# Autodesk Inventor assembly: 機体
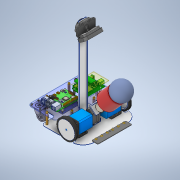
[picture p0: Inventor's stored thumbnail of the model, 180x180]
Saved by Autodesk Inventor 2020 (Build 240168000, 168)
## iProperties
Created: 2020-06-21
Part Number: 機体
Document SubType Name: Assembly
Designer: bsat3
Author: bsat3
## Documents named in this file (28)
- C:\Users\haya\Documents\Lecture\ロボット設計製作論４\2020\monotaro\IRC\機体.iam
- C:\Users\haya\Documents\Lecture\ロボット設計製作論４\2020\monotaro\IRC\知能ロボット\台車土台.ipt
- C:\Users\haya\Documents\Lecture\ロボット設計製作論４\2020\monotaro\IRC\モータ部分.iam
- C:\Users\haya\Documents\Lecture\ロボット設計製作論４\2020\monotaro\IRC\知能ロボット\知能ロボット吸引機構.iam
- C:\Users\haya\Documents\Lecture\ロボット設計製作論４\2020\monotaro\IRC\line_sensor.ipt
- C:\Users\haya\Documents\Lecture\ロボット設計製作論４\2020\monotaro\IRC\キャスタ.ipt
- C:\Users\haya\Documents\Lecture\ロボット設計製作論４\2020\monotaro\IRC\SBD-O3-25.ipt
- C:\Users\haya\Documents\Lecture\ロボット設計製作論４\2020\monotaro\IRC\arduino\arduino uno.iam
- C:\Users\haya\Documents\Lecture\ロボット設計製作論４\2020\monotaro\IRC\upper_frame.ipt
- C:\Users\haya\Documents\Lecture\ロボット設計製作論４\2020\monotaro\IRC\servo_motor\KRS2500_scale.ipt
- C:\Users\haya\Documents\Lecture\ロボット設計製作論４\2020\monotaro\IRC\fan_motor\Assembly 1.iam
- C:\Users\haya\Documents\Lecture\ロボット設計製作論４\2020\monotaro\IRC\arm.ipt
- C:\Users\haya\Documents\Lecture\ロボット設計製作論４\2020\monotaro\IRC\camera\CAMERA ASSEMBLY.iam
- C:\Users\haya\Documents\Lecture\ロボット設計製作論４\2020\monotaro\IRC\camera_stand.ipt
- C:\Users\haya\Documents\Lecture\ロボット設計製作論４\2020\monotaro\IRC\raspberrypi\Raspberry Pi 4 Model B.iam
- C:\Users\haya\Documents\Lecture\ロボット設計製作論４\2020\monotaro\IRC\battery_holder\1_5V_holder4AA.ipt
- C:\Users\haya\Documents\Lecture\ロボット設計製作論４\2020\monotaro\IRC\servo_arm.ipt
- C:\Users\haya\Documents\Lecture\ロボット設計製作論４\2020\monotaro\IRC\ball.ipt
- C:\Users\haya\Documents\Lecture\ロボット設計製作論４\2020\monotaro\IRC\servo_bracket.ipt
- C:\Users\haya\Documents\Lecture\ロボット設計製作論４\2020\monotaro\IRC\BOB-M3-2-3W.ipt
- C:\Users\haya\Documents\Lecture\ロボット設計製作論４\2020\monotaro\IRC\motor driver.ipt
- C:\Users\haya\Documents\Lecture\ロボット設計製作論４\2020\monotaro\IRC\shield.ipt
- C:\Users\haya\Documents\Lecture\ロボット設計製作論４\2020\monotaro\IRC\CSPELH-SUS-M3-5.ipt
- C:\Users\haya\Documents\Lecture\ロボット設計製作論４\2020\monotaro\IRC\CSPELH-SUS-M3-7.ipt
- C:\Users\haya\Documents\Lecture\ロボット設計製作論４\2020\monotaro\IRC\spacer_10mm.ipt
- C:\Users\haya\Documents\Lecture\ロボット設計製作論４\2020\monotaro\IRC\HNT1-ST-M3.ipt
- C:\Users\haya\Documents\Lecture\ロボット設計製作論４\2020\monotaro\IRC\CSPPN-ST-M3-6_203.ipt
- C:\Users\haya\Documents\Lecture\ロボット設計製作論４\2020\monotaro\IRC\E-6598.ipt
## Components (109 placed, 27 different names)
1. 台車土台:1 — メイト:3, フラッシュ:4, フラッシュ:5, メイト:5, メイト:6, メイト:7, メイト:8, 挿入:9, 挿入:10, 挿入:11, 挿入:12, 挿入:13, 挿入:14, フラッシュ:7, フラッシュ:8, メイト:13, メイト:18, フラッシュ:9, 挿入:32, 挿入:33, 挿入:42, 挿入:43, 挿入:48, 挿入:49, 挿入:50, 挿入:51, 挿入:52, 挿入:53, 挿入:54, 挿入:55, 挿入:56, 挿入:57, 挿入:58, 挿入:59, 挿入:60, 挿入:61, 挿入:62, 挿入:63, 挿入:64, 挿入:65, 挿入:66, 挿入:67, 挿入:68, 挿入:69, 挿入:70, 挿入:71, 挿入:72, 挿入:73, 挿入:74, 挿入:75
2. モータ部分:1 [sub-assembly] — フラッシュ:4, メイト:5, メイト:6
3. モータ部分:2 [sub-assembly] — フラッシュ:5, メイト:7, メイト:8
4. 知能ロボット吸引機構:1 [sub-assembly] — 挿入:24, 挿入:25, メイト:19, メイト:20
5. line_sensor:1 — 挿入:42, 挿入:43, 挿入:85, 挿入:86, 挿入:87, 挿入:88, 挿入:89, 挿入:90
6. キャスタ:1 — 挿入:15, 挿入:16, 挿入:34, 挿入:35, 挿入:36, 挿入:37
7. SBD-O3-25:1 — メイト:3, 挿入:9
8. arduino uno:1 [sub-assembly] — メイト:11, メイト:21, フラッシュ:10, フラッシュ:11, フラッシュ:16, フラッシュ:17, 挿入:81, 挿入:82, 挿入:83, 挿入:84
9. SBD-O3-25:2 — 挿入:10
10. SBD-O3-25:3 — 挿入:11
11. SBD-O3-25:4 — 挿入:12, メイト:10
12. SBD-O3-25:5 — 挿入:13
13. SBD-O3-25:6 — 挿入:14
14. upper_frame:1 — メイト:10, フラッシュ:7, 挿入:15, 挿入:16, 挿入:17, 挿入:18, フラッシュ:8, メイト:11, メイト:14, メイト:15, メイト:17, フラッシュ:16, フラッシュ:17, フラッシュ:18, フラッシュ:19, 挿入:91, 挿入:92, 挿入:93, 挿入:94, 挿入:95, 挿入:96, 挿入:97, 挿入:98, 挿入:99, 挿入:100, 挿入:101, 挿入:102, 挿入:103, 挿入:104, 挿入:105, 挿入:106, 挿入:107, 挿入:108, 挿入:109, 挿入:110, 挿入:111, 挿入:112
15. キャスタ:2 — 挿入:17, 挿入:18, 挿入:38, 挿入:39, 挿入:40, 挿入:41
16. KRS2500_scale:1 — 挿入:21, 挿入:26, 挿入:27
17. Assembly 1:1 [sub-assembly] — 挿入:19
18. arm:1 — 挿入:19, 挿入:22, 挿入:23, 挿入:24, 挿入:25
19. CAMERA ASSEMBLY:1 [sub-assembly] — メイト:16, メイト:24, 角度:1
20. camera_stand:1 — メイト:13, メイト:14, メイト:15, メイト:16, 挿入:44, 挿入:45, 挿入:46, 挿入:47, 挿入:113, 角度:1
21. Raspberry Pi 4 Model B:1 [sub-assembly] — メイト:17, フラッシュ:18, フラッシュ:19, 挿入:76, 挿入:77, 挿入:78, 挿入:79
22. 1_5V_holder4AA:1 — メイト:18, フラッシュ:9
23. servo_arm:1 — 挿入:21, 挿入:22, 挿入:23
24. ball:1 — メイト:19, メイト:20
25. servo_bracket:1 — 挿入:26, 挿入:27, 挿入:28, 挿入:29, 挿入:30, 挿入:31, 挿入:32, 挿入:33
26. BOB-M3-2-3W:1 — 挿入:28
27. BOB-M3-2-3W:2 — 挿入:29
28. BOB-M3-2-3W:3 — 挿入:30
29. BOB-M3-2-3W:4 — 挿入:31
30. BOB-M3-2-3W:5 — 挿入:34
31. BOB-M3-2-3W:6 — 挿入:35
32. BOB-M3-2-3W:7 — 挿入:36
33. BOB-M3-2-3W:8 — 挿入:37
34. BOB-M3-2-3W:9 — 挿入:38
35. BOB-M3-2-3W:10 — 挿入:39
36. BOB-M3-2-3W:11 — 挿入:41
37. BOB-M3-2-3W:12 — 挿入:40
38. motor driver:1 — メイト:23, フラッシュ:13, フラッシュ:15
39. motor driver:2 — メイト:22, フラッシュ:12, フラッシュ:14
40. shield:1 — メイト:21, フラッシュ:10, フラッシュ:11, メイト:22, フラッシュ:12, メイト:23, フラッシュ:13, フラッシュ:14, フラッシュ:15
41. BOB-M3-2-3W:13 — 挿入:44
42. BOB-M3-2-3W:14 — 挿入:45
43. BOB-M3-2-3W:15 — 挿入:46
44. BOB-M3-2-3W:16 — 挿入:47
45. CSPELH-SUS-M3-5:1 — 挿入:48
46. CSPELH-SUS-M3-5:2 — 挿入:49
47. CSPELH-SUS-M3-5:3 — 挿入:50
48. CSPELH-SUS-M3-5:4 — 挿入:51
49. CSPELH-SUS-M3-7:1 — 挿入:52
50. CSPELH-SUS-M3-7:2 — 挿入:53
51. CSPELH-SUS-M3-7:3 — 挿入:54
52. CSPELH-SUS-M3-7:4 — 挿入:55
53. CSPELH-SUS-M3-7:5 — 挿入:56
54. CSPELH-SUS-M3-7:6 — 挿入:58
55. CSPELH-SUS-M3-7:7 — 挿入:59
56. CSPELH-SUS-M3-7:8 — 挿入:57
57. CSPELH-SUS-M3-7:10 — 挿入:62
58. CSPELH-SUS-M3-7:11 — 挿入:61
59. CSPELH-SUS-M3-7:12 — 挿入:60
60. CSPELH-SUS-M3-7:13 — 挿入:63
61. CSPELH-SUS-M3-7:14 — 挿入:64
62. CSPELH-SUS-M3-7:15 — 挿入:65
63. CSPELH-SUS-M3-7:16 — 挿入:67
64. CSPELH-SUS-M3-7:17 — 挿入:66
65. CSPELH-SUS-M3-7:18 — 挿入:68
66. CSPELH-SUS-M3-7:19 — 挿入:72
67. CSPELH-SUS-M3-7:20 — 挿入:70
68. CSPELH-SUS-M3-7:21 — 挿入:71
69. CSPELH-SUS-M3-7:22 — 挿入:69
70. CSPELH-SUS-M3-7:23 — 挿入:75
71. CSPELH-SUS-M3-7:24 — 挿入:74
72. CSPELH-SUS-M3-7:25 — 挿入:73
73. spacer_10mm:1 — 挿入:78
74. spacer_10mm:2 — 挿入:79
75. spacer_10mm:3 — 挿入:77
76. spacer_10mm:4 — 挿入:76
77. spacer_10mm:6 — 挿入:81
78. spacer_10mm:7 — 挿入:83
79. spacer_10mm:8 — 挿入:82
80. spacer_10mm:9 — 挿入:84
81. HNT1-ST-M3:1 — 挿入:85
82. HNT1-ST-M3:2 — 挿入:90
83. HNT1-ST-M3:3 — 挿入:89
84. HNT1-ST-M3:4 — 挿入:88
85. HNT1-ST-M3:5 — 挿入:87
86. HNT1-ST-M3:6 — 挿入:86
87. HNT1-ST-M3:7 — 挿入:96
88. HNT1-ST-M3:8 — 挿入:94
89. HNT1-ST-M3:9 — 挿入:93
90. HNT1-ST-M3:10 — 挿入:95
91. HNT1-ST-M3:11 — 挿入:92
92. HNT1-ST-M3:12 — 挿入:91
93. CSPPN-ST-M3-6_203:1 — 挿入:97
94. CSPPN-ST-M3-6_203:2 — 挿入:98
95. CSPPN-ST-M3-6_203:3 — 挿入:99
96. CSPPN-ST-M3-6_203:4 — 挿入:100
97. CSPPN-ST-M3-6_203:5 — 挿入:101
98. CSPPN-ST-M3-6_203:6 — 挿入:102
99. CSPPN-ST-M3-6_203:7 — 挿入:103
100. CSPPN-ST-M3-6_203:8 — 挿入:104
101. CSPPN-ST-M3-6_203:9 — 挿入:105
102. CSPPN-ST-M3-6_203:10 — 挿入:108
103. CSPPN-ST-M3-6_203:11 — 挿入:107
104. CSPPN-ST-M3-6_203:12 — 挿入:106
105. CSPPN-ST-M3-6_203:13 — 挿入:109
106. CSPPN-ST-M3-6_203:14 — 挿入:110
107. CSPPN-ST-M3-6_203:15 — 挿入:111
108. CSPPN-ST-M3-6_203:16 — 挿入:112
109. E-6598:1 — 挿入:113, メイト:24
## Relationships (138: Insert 103, Mate 19, Flush 15, Angle 1)
- メイト:3 [Mate]: 台車土台:1 ↔ SBD-O3-25:1
- フラッシュ:4 [Flush]: 台車土台:1 ↔ モータ部分:1
- フラッシュ:5 [Flush]: 台車土台:1 ↔ モータ部分:2
- メイト:5 [Mate]: 台車土台:1 ↔ モータ部分:1
- メイト:6 [Mate] (-60 mm): 台車土台:1 ↔ モータ部分:1
- メイト:7 [Mate]: 台車土台:1 ↔ モータ部分:2
- メイト:8 [Mate] (-60 mm): 台車土台:1 ↔ モータ部分:2
- 挿入:9 [Insert]: 台車土台:1 ↔ SBD-O3-25:1
- 挿入:10 [Insert]: 台車土台:1 ↔ SBD-O3-25:2
- 挿入:11 [Insert]: 台車土台:1 ↔ SBD-O3-25:3
- 挿入:12 [Insert]: 台車土台:1 ↔ SBD-O3-25:4
- 挿入:13 [Insert]: 台車土台:1 ↔ SBD-O3-25:5
- 挿入:14 [Insert]: 台車土台:1 ↔ SBD-O3-25:6
- メイト:10 [Mate]: SBD-O3-25:4 ↔ upper_frame:1
- フラッシュ:7 [Flush]: 台車土台:1 ↔ upper_frame:1
- 挿入:15 [Insert]: キャスタ:1 ↔ upper_frame:1
- 挿入:16 [Insert]: キャスタ:1 ↔ upper_frame:1
- 挿入:17 [Insert]: upper_frame:1 ↔ キャスタ:2
- 挿入:18 [Insert]: upper_frame:1 ↔ キャスタ:2
- フラッシュ:8 [Flush]: 台車土台:1 ↔ upper_frame:1
- メイト:11 [Mate] (10 mm): arduino uno:1 ↔ upper_frame:1
- 挿入:19 [Insert]: Assembly 1:1 ↔ arm:1
- メイト:13 [Mate]: 台車土台:1 ↔ camera_stand:1
- メイト:14 [Mate]: upper_frame:1 ↔ camera_stand:1
- メイト:15 [Mate]: upper_frame:1 ↔ camera_stand:1
- メイト:16 [Mate]: CAMERA ASSEMBLY:1 ↔ camera_stand:1
- メイト:17 [Mate] (10 mm): upper_frame:1 ↔ Raspberry Pi 4 Model B:1
- メイト:18 [Mate]: 台車土台:1 ↔ 1_5V_holder4AA:1
- フラッシュ:9 [Flush]: 台車土台:1 ↔ 1_5V_holder4AA:1
- 挿入:21 [Insert] (3 mm): KRS2500_scale:1 ↔ servo_arm:1
- 挿入:22 [Insert]: arm:1 ↔ servo_arm:1
- 挿入:23 [Insert]: arm:1 ↔ servo_arm:1
- 挿入:24 [Insert]: 知能ロボット吸引機構:1 ↔ arm:1
- 挿入:25 [Insert]: 知能ロボット吸引機構:1 ↔ arm:1
- メイト:19 [Mate]: 知能ロボット吸引機構:1 ↔ ball:1
- メイト:20 [Mate] (16 mm): 知能ロボット吸引機構:1 ↔ ball:1
- 挿入:26 [Insert]: KRS2500_scale:1 ↔ servo_bracket:1
- 挿入:27 [Insert]: KRS2500_scale:1 ↔ servo_bracket:1
- 挿入:28 [Insert]: servo_bracket:1 ↔ BOB-M3-2-3W:1
- 挿入:29 [Insert]: servo_bracket:1 ↔ BOB-M3-2-3W:2
- 挿入:30 [Insert]: servo_bracket:1 ↔ BOB-M3-2-3W:3
- 挿入:31 [Insert]: servo_bracket:1 ↔ BOB-M3-2-3W:4
- 挿入:32 [Insert]: 台車土台:1 ↔ servo_bracket:1
- 挿入:33 [Insert]: 台車土台:1 ↔ servo_bracket:1
- 挿入:34 [Insert]: キャスタ:1 ↔ BOB-M3-2-3W:5
- 挿入:35 [Insert]: キャスタ:1 ↔ BOB-M3-2-3W:6
- 挿入:36 [Insert]: キャスタ:1 ↔ BOB-M3-2-3W:7
- 挿入:37 [Insert]: キャスタ:1 ↔ BOB-M3-2-3W:8
- 挿入:38 [Insert]: キャスタ:2 ↔ BOB-M3-2-3W:9
- 挿入:39 [Insert]: キャスタ:2 ↔ BOB-M3-2-3W:10
- 挿入:40 [Insert]: キャスタ:2 ↔ BOB-M3-2-3W:12
- 挿入:41 [Insert]: キャスタ:2 ↔ BOB-M3-2-3W:11
- 挿入:42 [Insert]: 台車土台:1 ↔ line_sensor:1
- 挿入:43 [Insert]: 台車土台:1 ↔ line_sensor:1
- メイト:21 [Mate] (3 mm): arduino uno:1 ↔ shield:1
- フラッシュ:10 [Flush]: arduino uno:1 ↔ shield:1
- フラッシュ:11 [Flush]: arduino uno:1 ↔ shield:1
- メイト:22 [Mate] (10 mm): motor driver:2 ↔ shield:1
- フラッシュ:12 [Flush] (4 mm): motor driver:2 ↔ shield:1
- メイト:23 [Mate] (10 mm): motor driver:1 ↔ shield:1
- フラッシュ:13 [Flush] (26 mm): motor driver:1 ↔ shield:1
- フラッシュ:14 [Flush] (6 mm): motor driver:2 ↔ shield:1
- フラッシュ:15 [Flush] (6 mm): motor driver:1 ↔ shield:1
- フラッシュ:16 [Flush] (14 mm): arduino uno:1 ↔ upper_frame:1
- フラッシュ:17 [Flush] (22 mm): arduino uno:1 ↔ upper_frame:1
- フラッシュ:18 [Flush] (30 mm): upper_frame:1 ↔ Raspberry Pi 4 Model B:1
- フラッシュ:19 [Flush] (20 mm): upper_frame:1 ↔ Raspberry Pi 4 Model B:1
- 挿入:44 [Insert]: camera_stand:1 ↔ BOB-M3-2-3W:13
- 挿入:45 [Insert]: camera_stand:1 ↔ BOB-M3-2-3W:14
- 挿入:46 [Insert]: camera_stand:1 ↔ BOB-M3-2-3W:15
- 挿入:47 [Insert]: camera_stand:1 ↔ BOB-M3-2-3W:16
- 挿入:48 [Insert]: 台車土台:1 ↔ CSPELH-SUS-M3-5:1
- 挿入:49 [Insert]: 台車土台:1 ↔ CSPELH-SUS-M3-5:2
- 挿入:50 [Insert]: 台車土台:1 ↔ CSPELH-SUS-M3-5:3
- 挿入:51 [Insert]: 台車土台:1 ↔ CSPELH-SUS-M3-5:4
- 挿入:52 [Insert]: 台車土台:1 ↔ CSPELH-SUS-M3-7:1
- 挿入:53 [Insert]: 台車土台:1 ↔ CSPELH-SUS-M3-7:2
- 挿入:54 [Insert]: 台車土台:1 ↔ CSPELH-SUS-M3-7:3
- 挿入:55 [Insert]: 台車土台:1 ↔ CSPELH-SUS-M3-7:4
- 挿入:56 [Insert]: 台車土台:1 ↔ CSPELH-SUS-M3-7:5
- 挿入:57 [Insert]: 台車土台:1 ↔ CSPELH-SUS-M3-7:8
- 挿入:58 [Insert]: 台車土台:1 ↔ CSPELH-SUS-M3-7:6
- 挿入:59 [Insert]: 台車土台:1 ↔ CSPELH-SUS-M3-7:7
- 挿入:60 [Insert]: 台車土台:1 ↔ CSPELH-SUS-M3-7:12
- 挿入:61 [Insert]: 台車土台:1 ↔ CSPELH-SUS-M3-7:11
- 挿入:62 [Insert]: 台車土台:1 ↔ CSPELH-SUS-M3-7:10
- 挿入:63 [Insert]: 台車土台:1 ↔ CSPELH-SUS-M3-7:13
- 挿入:64 [Insert]: 台車土台:1 ↔ CSPELH-SUS-M3-7:14
- 挿入:65 [Insert]: 台車土台:1 ↔ CSPELH-SUS-M3-7:15
- 挿入:66 [Insert]: 台車土台:1 ↔ CSPELH-SUS-M3-7:17
- 挿入:67 [Insert]: 台車土台:1 ↔ CSPELH-SUS-M3-7:16
- 挿入:68 [Insert]: 台車土台:1 ↔ CSPELH-SUS-M3-7:18
- 挿入:69 [Insert]: 台車土台:1 ↔ CSPELH-SUS-M3-7:22
- 挿入:70 [Insert]: 台車土台:1 ↔ CSPELH-SUS-M3-7:20
- 挿入:71 [Insert]: 台車土台:1 ↔ CSPELH-SUS-M3-7:21
- 挿入:72 [Insert]: 台車土台:1 ↔ CSPELH-SUS-M3-7:19
- 挿入:73 [Insert]: 台車土台:1 ↔ CSPELH-SUS-M3-7:25
- 挿入:74 [Insert]: 台車土台:1 ↔ CSPELH-SUS-M3-7:24
- 挿入:75 [Insert]: 台車土台:1 ↔ CSPELH-SUS-M3-7:23
- 挿入:76 [Insert]: Raspberry Pi 4 Model B:1 ↔ spacer_10mm:4
- 挿入:77 [Insert]: Raspberry Pi 4 Model B:1 ↔ spacer_10mm:3
- 挿入:78 [Insert]: Raspberry Pi 4 Model B:1 ↔ spacer_10mm:1
- 挿入:79 [Insert]: Raspberry Pi 4 Model B:1 ↔ spacer_10mm:2
- 挿入:81 [Insert]: arduino uno:1 ↔ spacer_10mm:6
- 挿入:82 [Insert]: arduino uno:1 ↔ spacer_10mm:8
- 挿入:83 [Insert]: arduino uno:1 ↔ spacer_10mm:7
- 挿入:84 [Insert]: arduino uno:1 ↔ spacer_10mm:9
- 挿入:85 [Insert]: line_sensor:1 ↔ HNT1-ST-M3:1
- 挿入:86 [Insert]: line_sensor:1 ↔ HNT1-ST-M3:6
- 挿入:87 [Insert]: line_sensor:1 ↔ HNT1-ST-M3:5
- 挿入:88 [Insert]: line_sensor:1 ↔ HNT1-ST-M3:4
- 挿入:89 [Insert]: line_sensor:1 ↔ HNT1-ST-M3:3
- 挿入:90 [Insert]: line_sensor:1 ↔ HNT1-ST-M3:2
- 挿入:91 [Insert]: upper_frame:1 ↔ HNT1-ST-M3:12
- 挿入:92 [Insert]: upper_frame:1 ↔ HNT1-ST-M3:11
- 挿入:93 [Insert]: upper_frame:1 ↔ HNT1-ST-M3:9
- 挿入:94 [Insert]: upper_frame:1 ↔ HNT1-ST-M3:8
- 挿入:95 [Insert]: upper_frame:1 ↔ HNT1-ST-M3:10
- 挿入:96 [Insert]: upper_frame:1 ↔ HNT1-ST-M3:7
- 挿入:97 [Insert]: upper_frame:1 ↔ CSPPN-ST-M3-6_203:1
- 挿入:98 [Insert]: upper_frame:1 ↔ CSPPN-ST-M3-6_203:2
- 挿入:99 [Insert]: upper_frame:1 ↔ CSPPN-ST-M3-6_203:3
- 挿入:100 [Insert]: upper_frame:1 ↔ CSPPN-ST-M3-6_203:4
- 挿入:101 [Insert]: upper_frame:1 ↔ CSPPN-ST-M3-6_203:5
- 挿入:102 [Insert]: upper_frame:1 ↔ CSPPN-ST-M3-6_203:6
- 挿入:103 [Insert]: upper_frame:1 ↔ CSPPN-ST-M3-6_203:7
- 挿入:104 [Insert]: upper_frame:1 ↔ CSPPN-ST-M3-6_203:8
- 挿入:105 [Insert]: upper_frame:1 ↔ CSPPN-ST-M3-6_203:9
- 挿入:106 [Insert]: upper_frame:1 ↔ CSPPN-ST-M3-6_203:12
- 挿入:107 [Insert]: upper_frame:1 ↔ CSPPN-ST-M3-6_203:11
- 挿入:108 [Insert]: upper_frame:1 ↔ CSPPN-ST-M3-6_203:10
- 挿入:109 [Insert]: upper_frame:1 ↔ CSPPN-ST-M3-6_203:13
- 挿入:110 [Insert]: upper_frame:1 ↔ CSPPN-ST-M3-6_203:14
- 挿入:111 [Insert]: upper_frame:1 ↔ CSPPN-ST-M3-6_203:15
- 挿入:112 [Insert]: upper_frame:1 ↔ CSPPN-ST-M3-6_203:16
- 挿入:113 [Insert]: camera_stand:1 ↔ E-6598:1
- メイト:24 [Mate]: CAMERA ASSEMBLY:1 ↔ E-6598:1
- 角度:1 [Angle] (-90 deg): CAMERA ASSEMBLY:1 ↔ camera_stand:1
